# Autodesk Inventor assembly: Assembly5
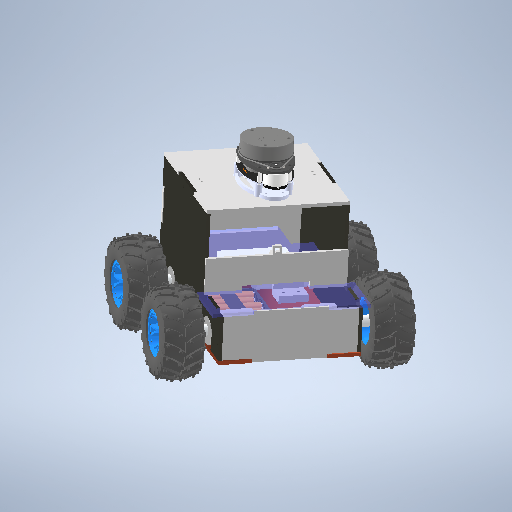
[picture p0: Inventor's stored thumbnail of the model, 512x512]
Saved by Autodesk Inventor 2025.3 (Build 293356030, 356C)
## iProperties
Created: 2026-06-28
Part Number: Assembly5
Document SubType Name: Assembly
Designer: user
Author: user
## Documents named in this file (11)
- C:\Docs\shcool\dojo\Design_3\Assembly5 - Copy.iam
- C:\Docs\shcool\dojo\Design_3\motor_wheel\wheel_base.iam
- C:\Docs\shcool\dojo\Design_3\battery_case\Battery_Housing_Full.iam
- C:\Docs\shcool\dojo\Design_3\chassis_boards\side.ipt
- C:\Docs\shcool\dojo\Design_3\chassis_boards\back.ipt
- C:\Docs\shcool\dojo\Design_3\chassis_boards\hood.ipt
- C:\Docs\shcool\dojo\Design_3\pi_internals\Complete_model.iam
- C:\Docs\shcool\dojo\Design_3\chassis_boards\cover.ipt
- C:\Docs\shcool\dojo\Design_3\chassis_boards\top.ipt
- C:\Docs\shcool\dojo\Design_3\lidar_assembly\assembled_lidar.iam
- C:\Docs\shcool\dojo\Design_3\chassis_boards\front.ipt
## Components (11 placed, 10 different names)
1. wheel_base:1 [sub-assembly] — Mate:1, Mate:4, Mate:5, Mate:6, Mate:17, Mate:18, Mate:24
2. Battery_Housing_Full:1 [sub-assembly] — Mate:1, Mate:24
3. side:1 — Mate:4, Mate:5, Mate:6, Mate:8, Mate:9, Mate:12, Mate:13, Mate:14, Mate:19, Mate:20, Mate:21, Mate:22
4. back:1 — Mate:8, Mate:9
5. hood:1 — Mate:16, Mate:19, Mate:20, Mate:25, Mate:26
6. Complete_model:1 [sub-assembly] — Mate:15, Mate:16
7. cover:1 — Mate:12, Mate:13, Mate:14, Mate:15
8. side:2 — Mate:17, Mate:18
9. top:1 — Mate:21, Mate:22, Mate:23
10. assembled_lidar:1 [sub-assembly] — Mate:23
11. front:1 — Mate:25, Mate:26
## Relationships (21: Mate 21)
- Mate:1: wheel_base:1 ↔ Battery_Housing_Full:1
- Mate:4: wheel_base:1 ↔ side:1
- Mate:5: wheel_base:1 ↔ side:1
- Mate:6: wheel_base:1 ↔ side:1
- Mate:8: side:1 ↔ back:1
- Mate:9: side:1 ↔ back:1
- Mate:12: side:1 ↔ cover:1
- Mate:13: side:1 ↔ cover:1
- Mate:14: side:1 ↔ cover:1
- Mate:15: Complete_model:1 ↔ cover:1
- Mate:16: hood:1 ↔ Complete_model:1
- Mate:17: wheel_base:1 ↔ side:2
- Mate:18: wheel_base:1 ↔ side:2
- Mate:19: side:1 ↔ hood:1
- Mate:20: side:1 ↔ hood:1
- Mate:21: side:1 ↔ top:1
- Mate:22: side:1 ↔ top:1
- Mate:23: top:1 ↔ assembled_lidar:1
- Mate:24: wheel_base:1 ↔ Battery_Housing_Full:1
- Mate:25: hood:1 ↔ front:1
- Mate:26: hood:1 ↔ front:1
